# Autodesk Inventor assembly: DoubleLengthCarrier
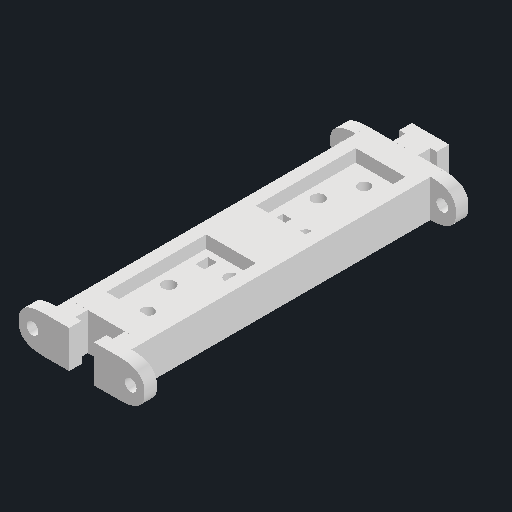
[picture p0: Inventor's stored thumbnail of the model, 512x512]
Saved by Autodesk Inventor 2024.1 (Build 281209000, 209)
## iProperties
Created: 2023-08-17
Part Number: DoubleLengthCarrier
Document SubType Name: Assembly
Designer: Eleanor
Author: Eleanor
## Documents named in this file (4)
- C:\Users\Eleanor\Documents\Inventor\4.5mm ERS\DoubleLengthCarrier.iam
- C:\Users\Eleanor\Documents\Inventor\4.5mm ERS\Connector_A.ipt
- C:\Users\Eleanor\Documents\Inventor\4.5mm ERS\Connector_B.ipt
- C:\Users\Eleanor\Documents\Inventor\4.5mm ERS\ExtendedSlottedCarrier.ipt
## Components (3 placed, 3 different names)
1. Connector_A:1 — Mate:1, Flush:1
2. Connector_B:1 — Flush:2, Flush:3
3. ExtendedSlottedCarrier:1 — Mate:1, Flush:1, Flush:2, Flush:3
## Relationships (4: Flush 3, Mate 1)
- Mate:1: Connector_A:1 ↔ ExtendedSlottedCarrier:1
- Flush:1: Connector_A:1 ↔ ExtendedSlottedCarrier:1
- Flush:2: Connector_B:1 ↔ ExtendedSlottedCarrier:1
- Flush:3: Connector_B:1 ↔ ExtendedSlottedCarrier:1
